# Autodesk Inventor assembly: Final Assembly - Plate Pouring III
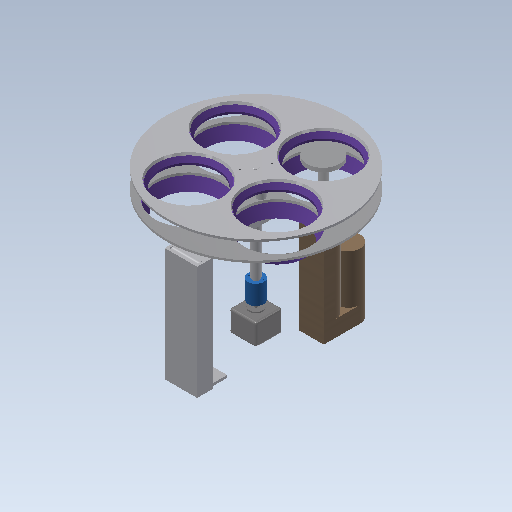
[picture p0: Inventor's stored thumbnail of the model, 512x512]
Saved by Autodesk Inventor 2021.3 (Build 253353010, 353A)
## iProperties
Created: 2015-11-30
Part Number: Final Assembly - Plate Pouring III
Document SubType Name: Assembly
Designer: zwrouse
Author: zwrouse
## Documents named in this file (18)
- C:\Users\Dell\Downloads\plate-pouring-system-1.snapshot.9\CAD Files\Final Assembly - Plate Pouring III.iam
- C:\Users\Dell\Downloads\plate-pouring-system-1.snapshot.9\CAD Files\NEMA Motor 17.ipt
- C:\Users\Dell\Downloads\plate-pouring-system-1.snapshot.9\CAD Files\Shaft Coupling.ipt
- C:\Users\Dell\Downloads\plate-pouring-system-1.snapshot.9\CAD Files\Short Axle.ipt
- C:\Users\Dell\Downloads\plate-pouring-system-1.snapshot.9\CAD Files\3-8 Washer.ipt
- C:\Users\Dell\Downloads\plate-pouring-system-1.snapshot.9\CAD Files\Base Stage.ipt
- C:\Users\Dell\Downloads\plate-pouring-system-1.snapshot.9\CAD Files\Imported Components\HEX NUT 3-8\HEX NUT 3-8.ipt
- C:\Users\Dell\Downloads\plate-pouring-system-1.snapshot.9\CAD Files\Lid Stage.ipt
- C:\Users\Dell\Downloads\plate-pouring-system-1.snapshot.9\CAD Files\base plate cone.ipt
- C:\Users\Dell\Downloads\plate-pouring-system-1.snapshot.9\CAD Files\Lid Cone.ipt
- C:\Users\Dell\Downloads\plate-pouring-system-1.snapshot.9\CAD Files\Stage Balancer.ipt
- C:\Users\Dell\Downloads\plate-pouring-system-1.snapshot.9\CAD Files\Imported Components\5-40 Screw\5-40 Screw.ipt
- C:\Users\Dell\Downloads\plate-pouring-system-1.snapshot.9\CAD Files\Short C.ipt
- C:\Users\Dell\Downloads\plate-pouring-system-1.snapshot.9\CAD Files\Small Bracket.ipt
- C:\Users\Dell\Downloads\plate-pouring-system-1.snapshot.9\CAD Files\Block.ipt
- C:\Users\Dell\Downloads\plate-pouring-system-1.snapshot.9\CAD Files\actuator.ipt
- C:\Users\Dell\Downloads\plate-pouring-system-1.snapshot.9\CAD Files\Peristaltic Pump.ipt
- C:\Users\Dell\Downloads\plate-pouring-system-1.snapshot.9\CAD Files\Actuator new.ipt
## Components (26 placed, 17 different names)
1. NEMA Motor 17:1 — Flush:1, Mate:1, Flush:2, Mate:2, Mate:3, Mate:4, Flush:6
2. Shaft Coupling:1 — Flush:2, Mate:2
3. Short Axle:1 — Mate:3, Mate:4, Mate:5, Mate:6, Mate:8, Mate:10, Flush:3, Mate:37, Mate:53
4. 3-8 Washer:1 — Mate:5, Mate:6, Mate:7
5. Base Stage:1 — Mate:7, Mate:8, Mate:9, Mate:13, Mate:14, Mate:15, Mate:16, Mate:19, Mate:34, Mate:36, Mate:40, Mate:41, Mate:42
6. HEX NUT 3-8:1 — Mate:9, Mate:10
7. Lid Stage:1 — Flush:3, Mate:20, Mate:21, Mate:22, Mate:23, Mate:24, Mate:25, Mate:26, Mate:27, Mate:28, Mate:29, Mate:31, Mate:37, Mate:38, Mate:39, Mate:40, Insert:16
8. base plate cone:1 — Mate:19, Mate:20
9. base plate cone:2 — Mate:41, Mate:42
10. base plate cone:3 — Mate:15, Mate:16
11. base plate cone:4 — Mate:13, Mate:14
12. Lid Cone:1 — Mate:23, Mate:24
13. Lid Cone:2 — Mate:21, Mate:22
14. Lid Cone:3 — Mate:25, Mate:26
15. Lid Cone:4 — Mate:27, Mate:28
16. Stage Balancer:1 — Mate:31, Mate:38, Mate:43
17. Stage Balancer:2 — Mate:29, Mate:33, Mate:39
18. 5-40 Screw:1 — Mate:33, Mate:34
19. 5-40 Screw:2 — Mate:36, Mate:43
20. Short C:1 — Flush:6, Mate:47, Mate:48, Mate:50, Flush:7, Flush:8, Flush:9
21. Small Bracket:1 — Mate:50, Flush:7, Flush:8, Mate:51, Mate:52
22. Small Bracket:2 — Mate:47, Mate:48
23. Block:1 — Flush:9, Mate:51, Mate:52, Mate:53
24. actuator:1 — Insert:16, Mate:101
25. Peristaltic Pump:1
26. Actuator new:1 — Mate:101
## Relationships (51: Mate 43, Flush 7, Insert 1)
- Flush:1: NEMA Motor 17:1
- Mate:1: NEMA Motor 17:1
- Flush:2: NEMA Motor 17:1 ↔ Shaft Coupling:1
- Mate:2: NEMA Motor 17:1 ↔ Shaft Coupling:1
- Mate:3: NEMA Motor 17:1 ↔ Short Axle:1
- Mate:4: NEMA Motor 17:1 ↔ Short Axle:1
- Mate:5: Short Axle:1 ↔ 3-8 Washer:1
- Mate:6: Short Axle:1 ↔ 3-8 Washer:1
- Mate:7: 3-8 Washer:1 ↔ Base Stage:1
- Mate:8: Short Axle:1 ↔ Base Stage:1
- Mate:9: Base Stage:1 ↔ HEX NUT 3-8:1
- Mate:10: Short Axle:1 ↔ HEX NUT 3-8:1
- Flush:3: Short Axle:1 ↔ Lid Stage:1
- Mate:13: Base Stage:1 ↔ base plate cone:4
- Mate:14: Base Stage:1 ↔ base plate cone:4
- Mate:15: Base Stage:1 ↔ base plate cone:3
- Mate:16: Base Stage:1 ↔ base plate cone:3
- Mate:19: Base Stage:1 ↔ base plate cone:1
- Mate:20: Lid Stage:1 ↔ base plate cone:1
- Mate:21: Lid Stage:1 ↔ Lid Cone:2
- Mate:22: Lid Stage:1 ↔ Lid Cone:2
- Mate:23: Lid Stage:1 ↔ Lid Cone:1
- Mate:24: Lid Stage:1 ↔ Lid Cone:1
- Mate:25: Lid Stage:1 ↔ Lid Cone:3
- Mate:26: Lid Stage:1 ↔ Lid Cone:3
- Mate:27: Lid Stage:1 ↔ Lid Cone:4
- Mate:28: Lid Stage:1 ↔ Lid Cone:4
- Mate:29: Lid Stage:1 ↔ Stage Balancer:2
- Mate:31: Lid Stage:1 ↔ Stage Balancer:1
- Mate:33: Stage Balancer:2 ↔ 5-40 Screw:1
- Mate:34: Base Stage:1 ↔ 5-40 Screw:1
- Mate:36: Base Stage:1 ↔ 5-40 Screw:2
- Mate:37: Short Axle:1 ↔ Lid Stage:1
- Mate:38: Lid Stage:1 ↔ Stage Balancer:1
- Mate:39: Lid Stage:1 ↔ Stage Balancer:2
- Mate:40: Base Stage:1 ↔ Lid Stage:1
- Mate:41: Base Stage:1 ↔ base plate cone:2
- Mate:42: Base Stage:1 ↔ base plate cone:2
- Mate:43: Stage Balancer:1 ↔ 5-40 Screw:2
- Flush:6 (-96.52 mm): NEMA Motor 17:1 ↔ Short C:1
- Mate:47: Short C:1 ↔ Small Bracket:2
- Mate:48: Short C:1 ↔ Small Bracket:2
- Mate:50: Short C:1 ↔ Small Bracket:1
- Flush:7: Short C:1 ↔ Small Bracket:1
- Flush:8: Short C:1 ↔ Small Bracket:1
- Flush:9 (25.4 mm): Short C:1 ↔ Block:1
- Mate:51: Small Bracket:1 ↔ Block:1
- Mate:52 (2.54 mm): Small Bracket:1 ↔ Block:1
- Mate:53: Short Axle:1 ↔ Block:1
- Insert:16: Lid Stage:1 ↔ actuator:1
- Mate:101: actuator:1 ↔ Actuator new:1
